# Autodesk Inventor assembly: Pomodoro Robot
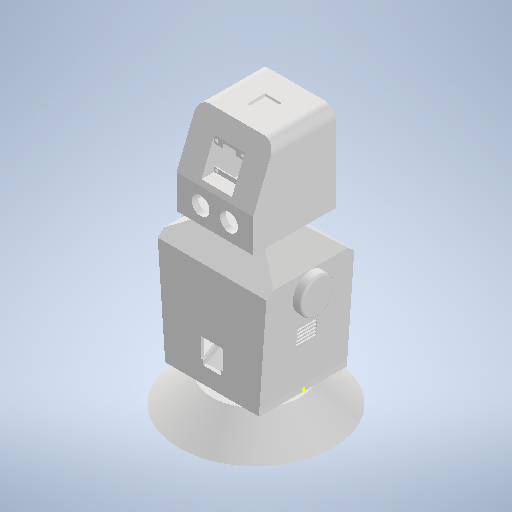
[picture p0: Inventor's stored thumbnail of the model, 512x512]
Saved by Autodesk Inventor 2025.3 (Build 293356030, 356C)
## iProperties
Created: 2026-07-19
Part Number: Pomodoro Robot
Document SubType Name: Assembly
Designer: Samuel Correa Vega
Author: Samuel Correa Vega
## Documents named in this file (10)
- C:\Users\Samuel Correa Vega\Documents\GitHub\Pomodoro_Robot\Design\Pomodoro Robot.iam
- C:\Users\Samuel Correa Vega\Documents\GitHub\Pomodoro_Robot\Design\Pomodoro Robot Head.ipt
- C:\Users\Samuel Correa Vega\Documents\GitHub\Pomodoro_Robot\Design\Pomodoro Robot Torso.ipt
- C:\Users\Samuel Correa Vega\Documents\GitHub\Pomodoro_Robot\Design\Pomodoro Robot Head's back.ipt
- C:\Users\Samuel Correa Vega\Documents\GitHub\Pomodoro_Robot\Design\BATTERY HOLDER x2.ipt
- C:\Users\Samuel Correa Vega\Documents\GitHub\Pomodoro_Robot\Design\Pomodoro Robot Torso's back.ipt
- C:\Users\Samuel Correa Vega\Documents\GitHub\Pomodoro_Robot\Design\Pomodoro Robot Base.ipt
- C:\Users\Samuel Correa Vega\Documents\GitHub\Pomodoro_Robot\Design\Pomodoro Robot Neck.ipt
- C:\Users\Samuel Correa Vega\Documents\GitHub\Pomodoro_Robot\Design\SG90 - Micro Servo 9g - Tower Pro.1.ipt
- C:\Users\Samuel Correa Vega\Documents\GitHub\Pomodoro_Robot\Design\Pomodoro Robot Servo's piece.ipt
## Components (9 placed, 9 different names)
1. Pomodoro Robot Head:1 — Mate:1, Flush:1, Mate:2, Angle:7, Mate:27, Mate:29
2. Pomodoro Robot Torso:1 — Mate:1, Flush:1, Angle:1, Mate:3, Mate:4, Mate:5, Mate:6, Mate:7, Angle:2, Angle:6, Angle:8, Mate:28, Angle:9, Mate:33
3. Pomodoro Robot Head's back:1 — Mate:2, Angle:7
4. BATTERY HOLDER x2:1 — Angle:1, Mate:3
5. Pomodoro Robot Torso's back:2 — Mate:19, Mate:20, Mate:21, Mate:22, Angle:5, Angle:6
6. Pomodoro Robot Base:1 — Mate:27, Angle:8
7. Pomodoro Robot Neck:1 — Mate:28, Mate:29
8. SG90 - Micro Servo 9g - Tower Pro.1:3 — Angle:9, Mate:31, Mate:32, Mate:33, Flush:2, Symmetry:1
9. Pomodoro Robot Servo's piece:1 — Mate:31, Mate:32, Symmetry:1
## Relationships (40: Mate 29, Angle 8, Flush 2, Symmetry 1)
- Mate:1: Pomodoro Robot Head:1 ↔ Pomodoro Robot Torso:1
- Flush:1: Pomodoro Robot Head:1 ↔ Pomodoro Robot Torso:1
- Mate:2: Pomodoro Robot Head:1 ↔ Pomodoro Robot Head's back:1
- Angle:1 (0 deg): Pomodoro Robot Torso:1 ↔ BATTERY HOLDER x2:1
- Mate:3: Pomodoro Robot Torso:1 ↔ BATTERY HOLDER x2:1
- Mate:4: Pomodoro Robot Torso:1
- Mate:5: Pomodoro Robot Torso:1
- Mate:6: Pomodoro Robot Torso:1
- Mate:7: Pomodoro Robot Torso:1
- Mate:8
- Mate:9
- Mate:10
- Angle:2 (0 deg): Pomodoro Robot Torso:1
- Mate:15
- Mate:16
- Mate:17
- Mate:18
- Angle:4 (0 deg)
- Mate:19: Pomodoro Robot Torso's back:2
- Mate:20: Pomodoro Robot Torso's back:2
- Mate:21: Pomodoro Robot Torso's back:2
- Mate:22: Pomodoro Robot Torso's back:2
- Mate:23
- Mate:24
- Mate:25
- Angle:5 (0 deg): Pomodoro Robot Torso's back:2
- Mate:26
- Angle:6 (0 deg): Pomodoro Robot Torso:1 ↔ Pomodoro Robot Torso's back:2
- Angle:7 (0 deg): Pomodoro Robot Head:1 ↔ Pomodoro Robot Head's back:1
- Mate:27: Pomodoro Robot Head:1 ↔ Pomodoro Robot Base:1
- Angle:8 (0 deg): Pomodoro Robot Torso:1 ↔ Pomodoro Robot Base:1
- Mate:28: Pomodoro Robot Torso:1 ↔ Pomodoro Robot Neck:1
- Mate:29: Pomodoro Robot Head:1 ↔ Pomodoro Robot Neck:1
- Angle:9 (0 deg): Pomodoro Robot Torso:1 ↔ SG90 - Micro Servo 9g - Tower Pro.1:3
- Mate:31: SG90 - Micro Servo 9g - Tower Pro.1:3 ↔ Pomodoro Robot Servo's piece:1
- Mate:32: SG90 - Micro Servo 9g - Tower Pro.1:3 ↔ Pomodoro Robot Servo's piece:1
- Mate:33: Pomodoro Robot Torso:1 ↔ SG90 - Micro Servo 9g - Tower Pro.1:3
- Flush:2 (1.5875 mm): SG90 - Micro Servo 9g - Tower Pro.1:3
- Symmetry:1: SG90 - Micro Servo 9g - Tower Pro.1:3 ↔ Pomodoro Robot Servo's piece:1
- Mate:34
